# Autodesk Inventor assembly: fiveHoles3segmentHexKeyHolder
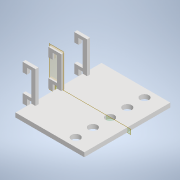
[picture p0: Inventor's stored thumbnail of the model, 180x180]
Saved by Autodesk Inventor 2020.2 (Build 242310000, 310)
## iProperties
Created: 2020-03-13
Part Number: fiveHoles3segmentHexKeyHolder
Document SubType Name: Assembly
Designer: robst
Author: robst
## Documents named in this file (3)
- C:\git\CAD-Development\robSteele\HouseProjects\Garage\Ikea\fiveHoles3segmentHexKeyHolder.iam
- C:\git\CAD-Development\robSteele\HouseProjects\Garage\Ikea\threeStartConfigurationV01.ipt
- C:\git\CAD-Development\robSteele\HouseProjects\Garage\Ikea\5-holes.ipt
## Components (2 placed, 2 different names)
1. threeStartConfigurationV01:1 — Mate:1, Flush:1, Flush:2
2. 5-holes:1 — Mate:1, Flush:1, Flush:2
## Relationships (3: Flush 2, Mate 1)
- Mate:1: threeStartConfigurationV01:1 ↔ 5-holes:1
- Flush:1: threeStartConfigurationV01:1 ↔ 5-holes:1
- Flush:2: threeStartConfigurationV01:1 ↔ 5-holes:1
